# Autodesk Inventor assembly: Arm 2.0 Assembly
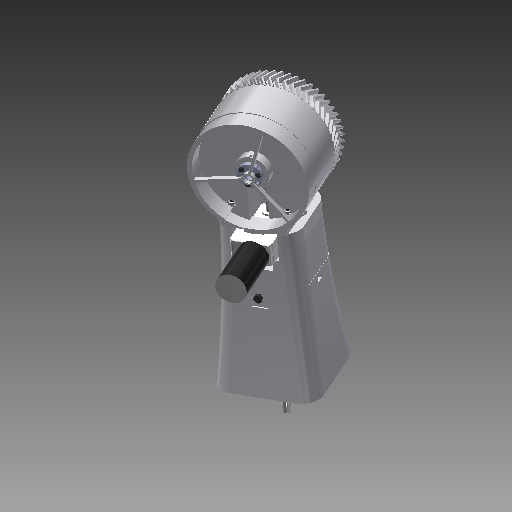
[picture p0: Inventor's stored thumbnail of the model, 512x512]
Saved by Autodesk Inventor 2017 (Build 210142000, 142)
## iProperties
Created: 2017-09-28
Part Number: Arm 2.0 Assembly
Document SubType Name: Assembly
Designer: Zach
Author: Zach
## Documents named in this file (17)
- C:\Users\Dell\Documents\GitHub\tr1\src\Body\Arm Assembly\Bicep Assembly\Bicep Assembly.iam
- C:\Users\Dell\Documents\GitHub\tr1\lib\8mm Hub.ipt
- C:\Users\Dell\Documents\GitHub\tr1\src\Body\Arm Assembly\Bicep Assembly\AA008c.ipt
- C:\Users\Dell\Documents\GitHub\tr1\src\Body\Arm Assembly\Arm Assembly\Design Accelerator\Spur Gears9.iam
- C:\Users\Dell\Documents\GitHub\tr1\lib\Content Center Files\R2017\en-US\ISO 4018\ISO 4018 - M5 x 25.ipt
- C:\Users\Dell\Documents\GitHub\tr1\lib\Content Center Files\R2017\en-US\ISO 7045  H\ISO 7045 - M3 x 12 - 4.8 - H - ISO.ipt
- C:\Users\Dell\Documents\GitHub\tr1\lib\Content Center Files\R2017\en-US\ISO 4018\ISO 4018 - M5 x 40.ipt
- C:\Users\Dell\Documents\GitHub\tr1\lib\Content Center Files\R2017\en-US\ISO 4035(2)\ISO 4035 - M5 - ISO.ipt
- C:\Users\Dell\Documents\GitHub\tr1\src\Body\Arm Assembly\Bicep Assembly\AA035c.ipt
- C:\Users\Dell\Documents\GitHub\tr1\src\Body\Arm Assembly\Bicep Assembly\AA008d2.ipt
- C:\Users\Dell\Documents\GitHub\tr1\lib\TSINY TS-42GZ495.ipt
- C:\Users\Dell\Documents\GitHub\tr1\lib\EMS22XXX-D28-LSX.ipt
- C:\Users\Dell\Documents\GitHub\tr1\src\Body\Arm Assembly\Bicep Assembly\AA052.ipt
- C:\Users\Dell\Documents\GitHub\tr1\src\Body\Arm Assembly\Bicep Assembly\AA054.ipt
- C:\Users\Dell\Documents\GitHub\tr1\lib\6mm Mounting Hub, thin.ipt
- C:\Users\Dell\Documents\GitHub\tr1\lib\8mm Mounting Hub, thin.ipt
- C:\Users\Dell\Documents\GitHub\tr1\src\Body\Arm Assembly\Bicep Assembly\AASG02b.ipt
## Components (31 placed, 16 different names)
1. AA008c:1 — Mate:1113, Mate:1114, Mate:1115, Mate:1125
2. AA008d2:1 — Mate:1104, Mate:1106, Mate:1107, Angle:22, Mate:1113, Mate:1114, Mate:1115, Mate:1124, Mate:1125, Mate:1157, Mate:1158, Mate:1159, Mate:1160, Mate:1161, Mate:1162, Mate:1163, Mate:1164, Mate:1165, Mate:1166, Mate:1170, Mate:1192, Mate:1193, Mate:1194, Mate:1195, Mate:1312
3. AA035c:1 — Mate:1167, Mate:1168, Mate:1169, Mate:1170, Mate:1171, Mate:1172, Mate:1173, Mate:1175, Angle:24, Angle:25, Mate:1176, Mate:1202, Mate:1203, Angle:1297, Mate:1312, Mate:1323, Mate:1324, Mate:1325
4. AA052:1 — Mate:1202
5. AA054:1 — Mate:1270, Flush:1272, Mate:1282, Mate:1320, Angle:1298
6. TSINY TS-42GZ495:3 — Mate:1104, Mate:1160, Mate:1161, Mate:1270, Flush:1272, Angle:1297, Angle:1298
7. 8mm Hub:6 — Mate:911, Mate:912, Mate:913, Mate:914, Mate:915, Mate:916, Mate:1203
8. EMS22XXX-D28-LSX:4 — Mate:1106, Mate:1107, Angle:22, Mate:1190, Mate:1313
9. AASG06 [sub-assembly] — Mate:1124, Mate:1190, Mate:1268, Mate:1269, Mate:1282, Mate:1314, Mate:1315, Mate:1321, Mate:1322
10. 6mm Mounting Hub, thin:1 — Mate:1313, Mate:1314, Mate:1315
11. ISO 7045 H M3 x 12 - 4.8 - H:10 — Mate:911, Mate:914
12. ISO 7045 H M3 x 12 - 4.8 - H:11 — Mate:913, Mate:915
13. ISO 7045 H M3 x 12 - 4.8 - H:12 — Mate:912, Mate:916
14. ISO 7045 H M3 x 12 - 4.8 - H:32 — Mate:1268, Mate:1269
15. ISO 4035 M5:1 — Mate:1167, Mate:1168
16. ISO 4035 M5:2 — Mate:852, Mate:1176
17. ISO 4035 M5:9 — Mate:1174, Mate:1175, Angle:24
18. ISO 4035 M5:10 — Mate:1027, Mate:1173, Angle:25
19. ISO 4018 M5 x 25:25 — Mate:1326, Mate:1329
20. ISO 4018 M5 x 25:27 — Mate:1328, Mate:1331
21. ISO 4018 M5 x 25:28 — Mate:1327, Mate:1330
22. ISO 4018 M5 x 25:29 — Mate:1157, Mate:1159
23. ISO 4018 M5 x 25:30 — Mate:1192, Mate:1193
24. ISO 4018 M5 x 25:31 — Mate:1194, Mate:1195
25. ISO 4018 M5 x 25:32 — Mate:1158
26. ISO 4018 M5 x 40:1 — Mate:1162, Mate:1169
27. ISO 4018 M5 x 40:2 — Mate:852, Mate:1163, Mate:1166
28. ISO 4018 M5 x 40:3 — Mate:1027, Mate:1165, Mate:1172
29. ISO 4018 M5 x 40:4 — Mate:1164, Mate:1171, Mate:1174
30. 8mm Mounting Hub, thin:1 — Mate:1320, Mate:1321, Mate:1322
31. AASG02b — Mate:1323, Mate:1324, Mate:1325, Mate:1326, Mate:1327, Mate:1328, Mate:1329, Mate:1330, Mate:1331
## Relationships (69: Mate 63, Angle 5, Flush 1)
- Mate:852: ISO 4035 M5:2 ↔ ISO 4018 M5 x 40:2
- Mate:911: 8mm Hub:6 ↔ ISO 7045 H M3 x 12 - 4.8 - H:10
- Mate:912: 8mm Hub:6 ↔ ISO 7045 H M3 x 12 - 4.8 - H:12
- Mate:913: 8mm Hub:6 ↔ ISO 7045 H M3 x 12 - 4.8 - H:11
- Mate:914: 8mm Hub:6 ↔ ISO 7045 H M3 x 12 - 4.8 - H:10
- Mate:915: 8mm Hub:6 ↔ ISO 7045 H M3 x 12 - 4.8 - H:11
- Mate:916: 8mm Hub:6 ↔ ISO 7045 H M3 x 12 - 4.8 - H:12
- Mate:1027: ISO 4035 M5:10 ↔ ISO 4018 M5 x 40:3
- Mate:1104: AA008d2:1 ↔ TSINY TS-42GZ495:3
- Mate:1106: AA008d2:1 ↔ EMS22XXX-D28-LSX:4
- Mate:1107: AA008d2:1 ↔ EMS22XXX-D28-LSX:4
- Angle:22 (0 deg): AA008d2:1 ↔ EMS22XXX-D28-LSX:4
- Mate:1113: AA008c:1 ↔ AA008d2:1
- Mate:1114: AA008c:1 ↔ AA008d2:1
- Mate:1115: AA008c:1 ↔ AA008d2:1
- Mate:1124: AA008d2:1 ↔ AASG06
- Mate:1125: AA008c:1 ↔ AA008d2:1
- Mate:1157: AA008d2:1 ↔ ISO 4018 M5 x 25:29
- Mate:1158: AA008d2:1 ↔ ISO 4018 M5 x 25:32
- Mate:1159: AA008d2:1 ↔ ISO 4018 M5 x 25:29
- Mate:1160: AA008d2:1 ↔ TSINY TS-42GZ495:3
- Mate:1161: AA008d2:1 ↔ TSINY TS-42GZ495:3
- Mate:1162: AA008d2:1 ↔ ISO 4018 M5 x 40:1
- Mate:1163: AA008d2:1 ↔ ISO 4018 M5 x 40:2
- Mate:1164: AA008d2:1 ↔ ISO 4018 M5 x 40:4
- Mate:1165: AA008d2:1 ↔ ISO 4018 M5 x 40:3
- Mate:1166: AA008d2:1 ↔ ISO 4018 M5 x 40:2
- Mate:1167: AA035c:1 ↔ ISO 4035 M5:1
- Mate:1168: AA035c:1 ↔ ISO 4035 M5:1
- Mate:1169: AA035c:1 ↔ ISO 4018 M5 x 40:1
- Mate:1170: AA008d2:1 ↔ AA035c:1
- Mate:1171: AA035c:1 ↔ ISO 4018 M5 x 40:4
- Mate:1172: AA035c:1 ↔ ISO 4018 M5 x 40:3
- Mate:1173: AA035c:1 ↔ ISO 4035 M5:10
- Mate:1174: ISO 4035 M5:9 ↔ ISO 4018 M5 x 40:4
- Mate:1175: AA035c:1 ↔ ISO 4035 M5:9
- Angle:24 (0 deg): AA035c:1 ↔ ISO 4035 M5:9
- Angle:25 (0 deg): AA035c:1 ↔ ISO 4035 M5:10
- Mate:1176: AA035c:1 ↔ ISO 4035 M5:2
- Mate:1190: EMS22XXX-D28-LSX:4 ↔ AASG06
- Mate:1192: AA008d2:1 ↔ ISO 4018 M5 x 25:30
- Mate:1193: AA008d2:1 ↔ ISO 4018 M5 x 25:30
- Mate:1194: AA008d2:1 ↔ ISO 4018 M5 x 25:31
- Mate:1195: AA008d2:1 ↔ ISO 4018 M5 x 25:31
- Mate:1202: AA035c:1 ↔ AA052:1
- Mate:1203: AA035c:1 ↔ 8mm Hub:6
- Mate:1268: AASG06 ↔ ISO 7045 H M3 x 12 - 4.8 - H:32
- Mate:1269: AASG06 ↔ ISO 7045 H M3 x 12 - 4.8 - H:32
- Mate:1270: AA054:1 ↔ TSINY TS-42GZ495:3
- Flush:1272: AA054:1 ↔ TSINY TS-42GZ495:3
- Mate:1282: AA054:1 ↔ AASG06
- Angle:1297 (0 deg): AA035c:1 ↔ TSINY TS-42GZ495:3
- Mate:1312: AA008d2:1 ↔ AA035c:1
- Mate:1313: EMS22XXX-D28-LSX:4 ↔ 6mm Mounting Hub, thin:1
- Mate:1314: AASG06 ↔ 6mm Mounting Hub, thin:1
- Mate:1315: AASG06 ↔ 6mm Mounting Hub, thin:1
- Mate:1320: AA054:1 ↔ 8mm Mounting Hub, thin:1
- Mate:1321: AASG06 ↔ 8mm Mounting Hub, thin:1
- Mate:1322: AASG06 ↔ 8mm Mounting Hub, thin:1
- Angle:1298 (0 deg): AA054:1 ↔ TSINY TS-42GZ495:3
- Mate:1323: AA035c:1 ↔ AASG02b
- Mate:1324: AA035c:1 ↔ AASG02b
- Mate:1325: AA035c:1 ↔ AASG02b
- Mate:1326: ISO 4018 M5 x 25:25 ↔ AASG02b
- Mate:1327: ISO 4018 M5 x 25:28 ↔ AASG02b
- Mate:1328: ISO 4018 M5 x 25:27 ↔ AASG02b
- Mate:1329: ISO 4018 M5 x 25:25 ↔ AASG02b
- Mate:1330: ISO 4018 M5 x 25:28 ↔ AASG02b
- Mate:1331: ISO 4018 M5 x 25:27 ↔ AASG02b
